# Autodesk Inventor assembly: Mellie Cart
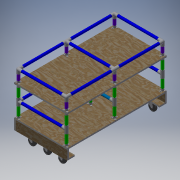
[picture p0: Inventor's stored thumbnail of the model, 180x180]
Saved by Autodesk Inventor 2018.2 (Build 222227000, 227)
## iProperties
Created: 2018-02-05
Part Number: Mellie Cart
Document SubType Name: Assembly
Designer: owner
Author: owner
## Documents named in this file (13)
- Z:\The Pickle - 4 - Copy\Final Carts\Mellie Cart\Mellie Cart.iam
- Z:\The Pickle - 4 - Copy\Final Carts\Mellie Cart\Mellie Plywood Base.ipt
- Z:\The Pickle - 4 - Copy\Final Carts\Stuff Used By All Carts\PVC Fittings (Formufit)\Wood Mount 1 Inch.ipt
- Z:\The Pickle - 4 - Copy\Final Carts\Stuff Used By All Carts\PVC Fittings (Formufit)\Tee 1 Inch.ipt
- Z:\The Pickle - 4 - Copy\Final Carts\Stuff Used By All Carts\PVC Fittings (Formufit)\4-way Tee 1 Inch.ipt
- Z:\The Pickle - 4 - Copy\Final Carts\Stuff Used By All Carts\PVC Fittings (Formufit)\5-way 1 Inch.ipt
- Z:\The Pickle - 4 - Copy\Final Carts\Stuff Used By All Carts\PVC Fittings (Formufit)\Cross 1 Inch.ipt
- Z:\The Pickle - 4 - Copy\Final Carts\Stuff Used By All Carts\PVC Fittings (Formufit)\3-way 90 1 Inch.ipt
- Z:\The Pickle - 4 - Copy\Final Carts\Mellie Cart\Mellie Pipe 1 (Main and Side).ipt
- Z:\The Pickle - 4 - Copy\Final Carts\Mellie Cart\Mellie Main Pipe 4.ipt
- Z:\The Pickle - 4 - Copy\Final Carts\Mellie Cart\Mellie Main Pipe 3.ipt
- Z:\The Pickle - 4 - Copy\Final Carts\Mellie Cart\Mellie Cart Wheel Mount.iam
- Z:\The Pickle - 4 - Copy\Final Carts\Mellie Cart\Mellie Main Pipe 2.ipt
## Components (69 placed, 12 different names)
1. Mellie Plywood Base:1 — Mate:1, Tangent:1, Tangent:2, Flush:7, Flush:8, Mate:17, Tangent:5, Tangent:6, Mate:18, Flush:30, Flush:31
2. Wood Mount 1 Inch:1 — Mate:1, Tangent:1, Tangent:2, Insert:1, Flush:6
3. Wood Mount 1 Inch:2 — Insert:7, Flush:5
4. Wood Mount 1 Inch:3 — Insert:29, Flush:4
5. Wood Mount 1 Inch:4 — Insert:30, Flush:3
6. Wood Mount 1 Inch:5 — Insert:31, Flush:2
7. Wood Mount 1 Inch:6 — Insert:32, Flush:1, Tangent:6
8. Wood Mount 1 Inch:7 — Insert:33, Mate:17, Tangent:5
9. Wood Mount 1 Inch:8 — Insert:34, Flush:5
10. Wood Mount 1 Inch:9 — Insert:35, Flush:4
11. Wood Mount 1 Inch:10 — Insert:36, Flush:6, Mate:2
12. Wood Mount 1 Inch:11 — Insert:37, Flush:3
13. Wood Mount 1 Inch:12 — Insert:38, Flush:2
14. Wood Mount 1 Inch:13 — Insert:39, Flush:1
15. Wood Mount 1 Inch:14 — Insert:40
16. Wood Mount 1 Inch:15 — Mate:3, Tangent:3, Tangent:4, Insert:41
17. Wood Mount 1 Inch:16 — Insert:56
18. Wood Mount 1 Inch:17 — Insert:57
19. Wood Mount 1 Inch:19 — Insert:59
20. Wood Mount 1 Inch:21 — Insert:61, Tangent:8
21. Wood Mount 1 Inch:25 — Insert:65, Tangent:7
22. Tee 1 Inch:1 — Insert:23, Insert:24, Insert:25
23. Tee 1 Inch:3 — Insert:14, Insert:15, Insert:17
24. Tee 1 Inch:4 — Insert:2, Insert:3, Insert:4
25. 4-way Tee 1 Inch:1 — Insert:21, Insert:22, Insert:26, Insert:27
26. 4-way Tee 1 Inch:2 — Insert:106, Insert:107, Insert:109, Insert:110
27. 4-way Tee 1 Inch:3 — Insert:5, Insert:6, Insert:8, Insert:28
28. 5-way 1 Inch:1 — Insert:9, Insert:10, Insert:11, Insert:19, Insert:20
29. Cross 1 Inch:1 — Insert:12, Insert:13, Insert:16, Insert:18
30. 3-way 90 1 Inch:1 — Insert:48, Insert:49, Insert:76
31. 3-way 90 1 Inch:4 — Insert:50, Insert:51, Insert:77
32. 3-way 90 1 Inch:5 — Insert:85, Insert:99, Insert:108
33. 3-way 90 1 Inch:6 — Insert:87, Insert:100, Insert:101
34. Mellie Pipe 1 (Main and Side):1 — Insert:22, Insert:23
35. Mellie Pipe 1 (Main and Side):2 — Insert:4, Insert:5
36. Mellie Pipe 1 (Main and Side):5 — Insert:49, Insert:50
37. Mellie Main Pipe 4:1 — Insert:28, Insert:34
38. Mellie Main Pipe 4:2 — Insert:26, Insert:32
39. Mellie Main Pipe 4:3 — Insert:18, Insert:37
40. Mellie Main Pipe 4:4 — Insert:16, Insert:30
41. Mellie Main Pipe 4:5 — Insert:15, Insert:31
42. Mellie Main Pipe 4:6 — Insert:25, Insert:40
43. Mellie Main Pipe 4:7 — Insert:24, Insert:33
44. Mellie Main Pipe 4:8 — Insert:10, Insert:29
45. Mellie Main Pipe 4:9 — Insert:17, Insert:38
46. Mellie Main Pipe 4:10 — Insert:3, Insert:36
47. Mellie Main Pipe 4:11 — Insert:6, Insert:7
48. Mellie Main Pipe 4:12 — Insert:19, Insert:35
49. Mellie Main Pipe 4:13 — Insert:1, Insert:2
50. Mellie Main Pipe 4:14 — Insert:27, Insert:39
51. Mellie Main Pipe 3:1 — Insert:11, Insert:12
52. Mellie Main Pipe 3:2 — Insert:13, Insert:14
53. Mellie Pipe 1 (Main and Side):8 — Insert:8, Insert:9
54. Mellie Pipe 1 (Main and Side):9 — Insert:51, Insert:110
55. Mellie Pipe 1 (Main and Side):10 — Insert:101, Insert:103
56. Mellie Pipe 1 (Main and Side):11 — Insert:48, Insert:104
57. Mellie Pipe 1 (Main and Side):12 — Insert:20, Insert:21
58. Mellie Main Pipe 2:1 — Insert:65, Insert:77
59. Mellie Main Pipe 2:2 — Insert:61, Insert:76
60. Mellie Main Pipe 2:3 — Insert:59, Insert:107
61. Mellie Main Pipe 2:4 — Insert:41, Insert:99
62. Mellie Main Pipe 2:5 — Insert:56, Insert:100
63. Mellie Main Pipe 2:6 — Insert:57, Insert:102
64. Mellie Plywood Base:2 — Mate:2, Flush:7, Flush:8, Mate:3, Tangent:3, Tangent:4, Tangent:7, Tangent:8
65. Mellie Pipe 1 (Main and Side):6 — Insert:85, Insert:87
66. 4-way Tee 1 Inch:4 — Insert:102, Insert:103, Insert:104, Insert:105
67. Mellie Pipe 1 (Main and Side):7 — Insert:105, Insert:106
68. Mellie Pipe 1 (Main and Side):13 — Insert:108, Insert:109
69. Mellie Cart Wheel Mount:1 [sub-assembly] — Mate:18, Flush:30, Flush:31
## Relationships (89: Insert 66, Flush 10, Tangent 8, Mate 5)
- Mate:1: Mellie Plywood Base:1 ↔ Wood Mount 1 Inch:1
- Tangent:1: Mellie Plywood Base:1 ↔ Wood Mount 1 Inch:1
- Tangent:2: Mellie Plywood Base:1 ↔ Wood Mount 1 Inch:1
- Insert:1: Wood Mount 1 Inch:1 ↔ Mellie Main Pipe 4:13
- Insert:2: Tee 1 Inch:4 ↔ Mellie Main Pipe 4:13
- Insert:3: Tee 1 Inch:4 ↔ Mellie Main Pipe 4:10
- Insert:4: Tee 1 Inch:4 ↔ Mellie Pipe 1 (Main and Side):2
- Insert:5: 4-way Tee 1 Inch:3 ↔ Mellie Pipe 1 (Main and Side):2
- Insert:6: 4-way Tee 1 Inch:3 ↔ Mellie Main Pipe 4:11
- Insert:7: Wood Mount 1 Inch:2 ↔ Mellie Main Pipe 4:11
- Insert:8: 4-way Tee 1 Inch:3 ↔ Mellie Pipe 1 (Main and Side):8
- Insert:9: 5-way 1 Inch:1 ↔ Mellie Pipe 1 (Main and Side):8
- Insert:10: 5-way 1 Inch:1 ↔ Mellie Main Pipe 4:8
- Insert:11: 5-way 1 Inch:1 ↔ Mellie Main Pipe 3:1
- Insert:12: Cross 1 Inch:1 ↔ Mellie Main Pipe 3:1
- Insert:13: Cross 1 Inch:1 ↔ Mellie Main Pipe 3:2
- Insert:14: Tee 1 Inch:3 ↔ Mellie Main Pipe 3:2
- Insert:15: Tee 1 Inch:3 ↔ Mellie Main Pipe 4:5
- Insert:16: Cross 1 Inch:1 ↔ Mellie Main Pipe 4:4
- Insert:17: Tee 1 Inch:3 ↔ Mellie Main Pipe 4:9
- Insert:18: Cross 1 Inch:1 ↔ Mellie Main Pipe 4:3
- Insert:19: 5-way 1 Inch:1 ↔ Mellie Main Pipe 4:12
- Insert:20: 5-way 1 Inch:1 ↔ Mellie Pipe 1 (Main and Side):12
- Insert:21: 4-way Tee 1 Inch:1 ↔ Mellie Pipe 1 (Main and Side):12
- Insert:22: 4-way Tee 1 Inch:1 ↔ Mellie Pipe 1 (Main and Side):1
- Insert:23: Tee 1 Inch:1 ↔ Mellie Pipe 1 (Main and Side):1
- Insert:24: Tee 1 Inch:1 ↔ Mellie Main Pipe 4:7
- Insert:25: Tee 1 Inch:1 ↔ Mellie Main Pipe 4:6
- Insert:26: 4-way Tee 1 Inch:1 ↔ Mellie Main Pipe 4:2
- Insert:27: 4-way Tee 1 Inch:1 ↔ Mellie Main Pipe 4:14
- Insert:28: 4-way Tee 1 Inch:3 ↔ Mellie Main Pipe 4:1
- Insert:29: Wood Mount 1 Inch:3 ↔ Mellie Main Pipe 4:8
- Insert:30: Wood Mount 1 Inch:4 ↔ Mellie Main Pipe 4:4
- Insert:31: Wood Mount 1 Inch:5 ↔ Mellie Main Pipe 4:5
- Insert:32: Wood Mount 1 Inch:6 ↔ Mellie Main Pipe 4:2
- Insert:33: Wood Mount 1 Inch:7 ↔ Mellie Main Pipe 4:7
- Insert:34: Wood Mount 1 Inch:8 ↔ Mellie Main Pipe 4:1
- Insert:35: Wood Mount 1 Inch:9 ↔ Mellie Main Pipe 4:12
- Insert:36: Wood Mount 1 Inch:10 ↔ Mellie Main Pipe 4:10
- Insert:37: Wood Mount 1 Inch:11 ↔ Mellie Main Pipe 4:3
- Insert:38: Wood Mount 1 Inch:12 ↔ Mellie Main Pipe 4:9
- Insert:39: Wood Mount 1 Inch:13 ↔ Mellie Main Pipe 4:14
- Insert:40: Wood Mount 1 Inch:14 ↔ Mellie Main Pipe 4:6
- Flush:1: Wood Mount 1 Inch:6 ↔ Wood Mount 1 Inch:13
- Flush:2: Wood Mount 1 Inch:5 ↔ Wood Mount 1 Inch:12
- Flush:3: Wood Mount 1 Inch:4 ↔ Wood Mount 1 Inch:11
- Flush:4: Wood Mount 1 Inch:3 ↔ Wood Mount 1 Inch:9
- Flush:5: Wood Mount 1 Inch:2 ↔ Wood Mount 1 Inch:8
- Flush:6: Wood Mount 1 Inch:1 ↔ Wood Mount 1 Inch:10
- Mate:2: Wood Mount 1 Inch:10 ↔ Mellie Plywood Base:2
- Flush:7: Mellie Plywood Base:1 ↔ Mellie Plywood Base:2
- Flush:8: Mellie Plywood Base:1 ↔ Mellie Plywood Base:2
- Mate:3: Wood Mount 1 Inch:15 ↔ Mellie Plywood Base:2
- Tangent:3: Wood Mount 1 Inch:15 ↔ Mellie Plywood Base:2
- Tangent:4: Wood Mount 1 Inch:15 ↔ Mellie Plywood Base:2
- Insert:41: Wood Mount 1 Inch:15 ↔ Mellie Main Pipe 2:4
- Insert:48: 3-way 90 1 Inch:1 ↔ Mellie Pipe 1 (Main and Side):11
- Insert:49: 3-way 90 1 Inch:1 ↔ Mellie Pipe 1 (Main and Side):5
- Insert:50: 3-way 90 1 Inch:4 ↔ Mellie Pipe 1 (Main and Side):5
- Insert:51: 3-way 90 1 Inch:4 ↔ Mellie Pipe 1 (Main and Side):9
- Insert:56: Wood Mount 1 Inch:16 ↔ Mellie Main Pipe 2:5
- Insert:57: Wood Mount 1 Inch:17 ↔ Mellie Main Pipe 2:6
- Insert:59: Wood Mount 1 Inch:19 ↔ Mellie Main Pipe 2:3
- Insert:61: Wood Mount 1 Inch:21 ↔ Mellie Main Pipe 2:2
- Insert:65: Wood Mount 1 Inch:25 ↔ Mellie Main Pipe 2:1
- Insert:76: 3-way 90 1 Inch:1 ↔ Mellie Main Pipe 2:2
- Insert:77: 3-way 90 1 Inch:4 ↔ Mellie Main Pipe 2:1
- Insert:85: 3-way 90 1 Inch:5 ↔ Mellie Pipe 1 (Main and Side):6
- Insert:87: 3-way 90 1 Inch:6 ↔ Mellie Pipe 1 (Main and Side):6
- Insert:99: 3-way 90 1 Inch:5 ↔ Mellie Main Pipe 2:4
- Insert:100: 3-way 90 1 Inch:6 ↔ Mellie Main Pipe 2:5
- Insert:101: 3-way 90 1 Inch:6 ↔ Mellie Pipe 1 (Main and Side):10
- Insert:102: Mellie Main Pipe 2:6 ↔ 4-way Tee 1 Inch:4
- Insert:103: Mellie Pipe 1 (Main and Side):10 ↔ 4-way Tee 1 Inch:4
- Insert:104: Mellie Pipe 1 (Main and Side):11 ↔ 4-way Tee 1 Inch:4
- Insert:105: 4-way Tee 1 Inch:4 ↔ Mellie Pipe 1 (Main and Side):7
- Insert:106: 4-way Tee 1 Inch:2 ↔ Mellie Pipe 1 (Main and Side):7
- Insert:107: 4-way Tee 1 Inch:2 ↔ Mellie Main Pipe 2:3
- Insert:108: 3-way 90 1 Inch:5 ↔ Mellie Pipe 1 (Main and Side):13
- Insert:109: 4-way Tee 1 Inch:2 ↔ Mellie Pipe 1 (Main and Side):13
- Insert:110: 4-way Tee 1 Inch:2 ↔ Mellie Pipe 1 (Main and Side):9
- Mate:17: Mellie Plywood Base:1 ↔ Wood Mount 1 Inch:7
- Tangent:5: Mellie Plywood Base:1 ↔ Wood Mount 1 Inch:7
- Tangent:6: Mellie Plywood Base:1 ↔ Wood Mount 1 Inch:6
- Mate:18: Mellie Plywood Base:1 ↔ Mellie Cart Wheel Mount:1
- Flush:30: Mellie Plywood Base:1 ↔ Mellie Cart Wheel Mount:1
- Flush:31: Mellie Plywood Base:1 ↔ Mellie Cart Wheel Mount:1
- Tangent:7: Wood Mount 1 Inch:25 ↔ Mellie Plywood Base:2
- Tangent:8: Wood Mount 1 Inch:21 ↔ Mellie Plywood Base:2
